# Autodesk Inventor assembly: s-assy-blacket2
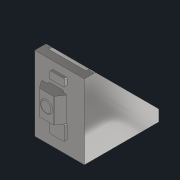
[picture p0: Inventor's stored thumbnail of the model, 180x180]
Saved by Autodesk Inventor 2022 (Build 260153000, 153)
## iProperties
Created: 2021-10-20
Part Number: s-assy-blacket2
Document SubType Name: Assembly
Designer: Yuta Kage
Author: Yuta Kage
## Documents named in this file (4)
- C:\Users\yuta0\Documents\GitHub\catchrobo_hardware\assy-scara\s-assy-blacket2.iam
- C:\Users\yuta0\Documents\GitHub\catchrobo_hardware\assy-scara\HBLFSNK5h5.ipt
- C:\Users\yuta0\Documents\GitHub\catchrobo_hardware\assy-shooter\HNTT5-5.ipt
- C:\Users\yuta0\Documents\GitHub\catchrobo_hardware\assy-shooter\CB5_10.ipt
## Components (3 placed, 3 different names)
1. HBLFSNK5h5:1 — メイト:1, メイト:2, メイト:4, 角度:1
2. HNTT5-5:1 — メイト:3, メイト:4, 角度:1
3. CB5_10:1 — メイト:1, メイト:2, メイト:3
## Relationships (5: Mate 4, Angle 1)
- メイト:1 [Mate]: HBLFSNK5h5:1 ↔ CB5_10:1
- メイト:2 [Mate]: HBLFSNK5h5:1 ↔ CB5_10:1
- メイト:3 [Mate]: HNTT5-5:1 ↔ CB5_10:1
- メイト:4 [Mate] (2 mm): HBLFSNK5h5:1 ↔ HNTT5-5:1
- 角度:1 [Angle] (0 deg): HBLFSNK5h5:1 ↔ HNTT5-5:1
